# Autodesk Inventor assembly: SteelM-StarS_MIR
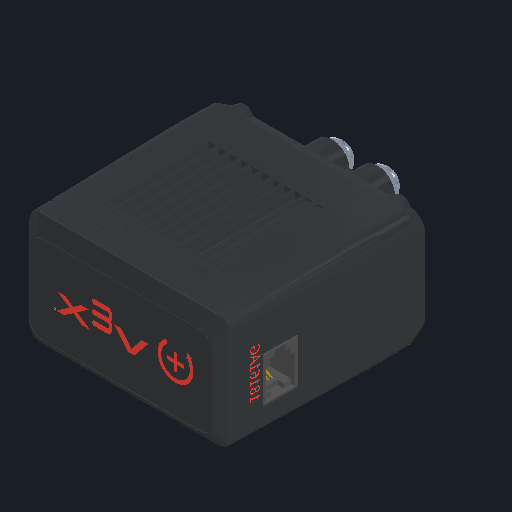
[picture p0: Inventor's stored thumbnail of the model, 512x512]
Saved by Autodesk Inventor 2024 (Build 280153000, 153)
## iProperties
Created: 2022-08-18
Part Number: SteelM-StarS_MIR
Document SubType Name: Assembly
Designer: avere
Author: ylu12
## Documents named in this file (4)
- C:\Users\avere\Documents\rbp_cad\zoomba_v0.3\chassis\mirrored_parts\SteelM-StarS_MIR.iam
- C:\Users\avere\Documents\rbp_cad\zoomba_v0.3\chassis\mirrored_parts\V5 Motor_MIR.ipt
- C:\Users\avere\Documents\rbp_cad\VEX-CAD-Inventor-1.41\Structure\Hardware\Screw Steel - Star\SScrew Star Smooth .500.ipt
- C:\Users\avere\Documents\rbp_cad\VEX-CAD-Inventor-1.41\Structure\Hardware\Screw Steel - Star.ipt
## Components (3 placed, 2 different names)
1. V5 Motor_MIR:1
2. SScrew Star Smooth .500:1
3. SScrew Star Smooth .500:2
## Named parameters: Thickness = 1.1938 mm
